# Autodesk Inventor assembly: foot_with_cleat
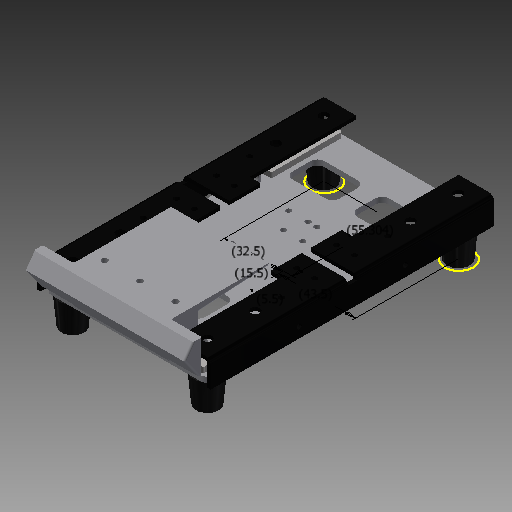
[picture p0: Inventor's stored thumbnail of the model, 512x512]
Saved by Autodesk Inventor 2018 (Build 220112000, 112)
## iProperties
Created: 2018-05-01
Part Number: foot_with_cleat
Document SubType Name: Assembly
Designer: medrimonia
Author: medrimonia
## Documents named in this file (6)
- C:\Users\etd\Dropbox\SigmaBan\SigmaBanV2.1\foot_with_cleat.iam
- C:\Users\etd\Dropbox\SigmaBan\SigmaBanV2.1\foot_sigmaban_plus.ipt
- C:\Users\etd\Dropbox\SigmaBan\SigmaBanV2.1\gauge_with_cleat.iam
- C:\Users\etd\Dropbox\SigmaBan\SigmaBanV2.1\protection_pied_sigmabanV2.ipt
- C:\Users\etd\Dropbox\SigmaBan\SigmaBanV2.1\external\M3_cube_standoff.ipt
- C:\Users\etd\Dropbox\SigmaBan\SigmaBanV2.1\gauge_protection_lateral.ipt
## Components (12 placed, 5 different names)
1. foot_sigmaban_plus:1 — Mate:1, Mate:2, Mate:3, Mate:4, Mate:5, Mate:6, Mate:7, Mate:8, Mate:9, Mate:10, Mate:11, Mate:12, Flush:2, Flush:3, Mate:17, Mate:18, Mate:19, Mate:20, Mate:21, Angle:1, Mate:22, Mate:23, Mate:27, Mate:28, Mate:29, Mate:30, Angle:2
2. gauge_with_cleat:1 [sub-assembly] — Mate:1, Mate:7, Mate:11
3. gauge_with_cleat:2 [sub-assembly] — Mate:4, Mate:5, Mate:10
4. gauge_with_cleat:3 [sub-assembly] — Mate:2, Mate:6, Mate:12, Mate:13
5. gauge_with_cleat:4 [sub-assembly] — Mate:3, Mate:8, Mate:9
6. protection_pied_sigmabanV2:1 — Mate:17, Mate:18, Mate:19
7. M3_cube_standoff:1 — Mate:20, Mate:21, Angle:1, Flush:4, Mate:24, Mate:25
8. M3_cube_standoff:2 — Mate:22, Mate:23, Flush:4, Mate:26
9. gauge_protection_lateral:1 — Mate:24, Mate:25, Mate:26
10. gauge_protection_lateral:2 — Mate:31, Mate:32, Mate:33
11. M3_cube_standoff:3 — Mate:28, Mate:30, Flush:5, Mate:33
12. M3_cube_standoff:4 — Mate:27, Mate:29, Angle:2, Flush:5, Mate:31, Mate:32
## Relationships (39: Mate 33, Flush 4, Angle 2)
- Mate:1: foot_sigmaban_plus:1 ↔ gauge_with_cleat:1
- Mate:2: foot_sigmaban_plus:1 ↔ gauge_with_cleat:3
- Mate:3: foot_sigmaban_plus:1 ↔ gauge_with_cleat:4
- Mate:4: foot_sigmaban_plus:1 ↔ gauge_with_cleat:2
- Mate:5: foot_sigmaban_plus:1 ↔ gauge_with_cleat:2
- Mate:6: foot_sigmaban_plus:1 ↔ gauge_with_cleat:3
- Mate:7: foot_sigmaban_plus:1 ↔ gauge_with_cleat:1
- Mate:8: foot_sigmaban_plus:1 ↔ gauge_with_cleat:4
- Mate:9: foot_sigmaban_plus:1 ↔ gauge_with_cleat:4
- Mate:10: foot_sigmaban_plus:1 ↔ gauge_with_cleat:2
- Mate:11: foot_sigmaban_plus:1 ↔ gauge_with_cleat:1
- Mate:12: foot_sigmaban_plus:1 ↔ gauge_with_cleat:3
- Flush:2: foot_sigmaban_plus:1
- Flush:3: foot_sigmaban_plus:1
- Mate:13: gauge_with_cleat:3
- Mate:14
- Mate:15
- Mate:16
- Mate:17: foot_sigmaban_plus:1 ↔ protection_pied_sigmabanV2:1
- Mate:18: foot_sigmaban_plus:1 ↔ protection_pied_sigmabanV2:1
- Mate:19: foot_sigmaban_plus:1 ↔ protection_pied_sigmabanV2:1
- Mate:20: foot_sigmaban_plus:1 ↔ M3_cube_standoff:1
- Mate:21: foot_sigmaban_plus:1 ↔ M3_cube_standoff:1
- Angle:1 (0 deg): foot_sigmaban_plus:1 ↔ M3_cube_standoff:1
- Mate:22: foot_sigmaban_plus:1 ↔ M3_cube_standoff:2
- Mate:23: foot_sigmaban_plus:1 ↔ M3_cube_standoff:2
- Flush:4: M3_cube_standoff:1 ↔ M3_cube_standoff:2
- Mate:24: M3_cube_standoff:1 ↔ gauge_protection_lateral:1
- Mate:25: M3_cube_standoff:1 ↔ gauge_protection_lateral:1
- Mate:26: M3_cube_standoff:2 ↔ gauge_protection_lateral:1
- Mate:27: foot_sigmaban_plus:1 ↔ M3_cube_standoff:4
- Mate:28: foot_sigmaban_plus:1 ↔ M3_cube_standoff:3
- Mate:29: foot_sigmaban_plus:1 ↔ M3_cube_standoff:4
- Mate:30: foot_sigmaban_plus:1 ↔ M3_cube_standoff:3
- Angle:2 (0 deg): foot_sigmaban_plus:1 ↔ M3_cube_standoff:4
- Flush:5: M3_cube_standoff:3 ↔ M3_cube_standoff:4
- Mate:31: gauge_protection_lateral:2 ↔ M3_cube_standoff:4
- Mate:32: gauge_protection_lateral:2 ↔ M3_cube_standoff:4
- Mate:33: gauge_protection_lateral:2 ↔ M3_cube_standoff:3
